# Autodesk Inventor assembly: 5267300 AEN-S-6-5-I-A---(0_high)
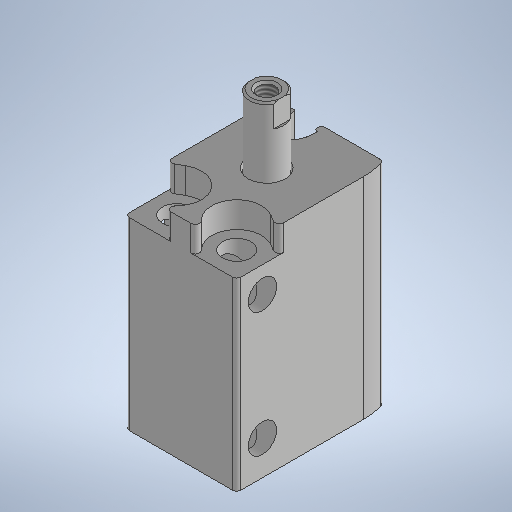
[picture p0: Inventor's stored thumbnail of the model, 512x512]
Saved by Autodesk Inventor 2025.2 (Build 292293000, 293)
## iProperties
Category: PARTsolutions
Company: FESTO
Created: 2025-06-16
Part Number: 5267300 AEN-S-6-5-I-A---(0_high)
Catalog Web Link: www.cadenas.de
Description: AEN-S-Compact cylinder
Vendor: FESTO
Document SubType Name: Assembly
Designer: psAdmin
Manufacturer: FESTO
Mass: 10.9 g
Surface Area: 34.4822 cm^2
Volume: 4.48385 cm^3
Density: 2.43095 g/cm^3
PSOL_IDENT_0: {ATYP=ASSISTANT},{DATA=script=$CADENAS_DATA/23d-libs/festo/webfesto.vbb&M_FAMILY=AEN&M_GROUP=01&M_PA
PSOL_IDENT_1: RTNO=5267300&IDCODE1=AEN-S-6-5-I-A&IDCODE2=&customer_number_cns=&MATES=1&LOD=HI&LOCKERP=0&SINGLEPART=
PSOL_IDENT_2: 1}
NB: 5267300 AEN-S-6-5-I-A---(0_high)
NN: AEN-S
NT: Compact cylinder
NBSYN: $TNR. $TYP.---($HUBST._$LODLEVEL.)
LINA: 5267300 AEN-S-6-5-I-A
CATALOG: Festo
TNR: 5267300
TYP: AEN-S-6-5-I-A
LODLEVEL: High
KDM: 6
HUB: 5
HUBST: 0
GA: I
DAF: P
AFF: A
A: 0
AF: 5
BG: 0
D1: 5.8
D2: 3.3
DA: 0
E1: 13
E2: 17.5
EE: M3
KF: M2.5
KK: -
L3: 10
L4: 7
LA: 0
MM: 4
P1: 6
P2: 4
P3: 3
PL1: 7
PL2: 3
RR: 0
RT: -
SF: 3.5
T: 3
T4: 0
TG: 7
WH: 3
WL: 2.7
ZA: 24.5
ZB: 27.5
CNSMASSEXACT: 0.0109
GTIN: 4052568422400
SUPPLIER: FESTO
ARTICLENO: 5267300 AEN-S-6-5-I-A---(0_high)
BOMINFO: 5267300 AEN-S-6-5-I-A
CREATOR: CADENAS GmbH
Title: 5267300 AEN-S-6-5-I-A
Author: Cadenas PARTsolutions
Comments: Compact cylinder
## Documents named in this file (3)
- C:\Users\Jakob\Documents\Kooperatives Studium HHN\Studium\3. Semester\CAD_Konstruktion - Schillo Paspa\Festo\AIS2024\5267300 AEN-S-6-5-I-A---(0_high).iam
- C:\Users\Jakob\Documents\Kooperatives Studium HHN\Studium\3. Semester\CAD_Konstruktion - Schillo Paspa\Festo\AIS2024\5267300 AEN-S-6-5-I-A---(highH).ipt
- C:\Users\Jakob\Documents\Kooperatives Studium HHN\Studium\3. Semester\CAD_Konstruktion - Schillo Paspa\Festo\AIS2024\5267300 AEN-S-6-5-I-A---(highP).ipt
## Components (2 placed, 2 different names)
1. 5267300 AEN-S-6-5-I-A---(highH):1 — TO_P_XY@1 <-> ANBAU_XY@2, TO_P_Z@1 <-> ANBAU_Z@2, TO_P_YZ@1 <-> ANBAU_YZ@2
2. 5267300 AEN-S-6-5-I-A---(highP):1 — TO_P_XY@1 <-> ANBAU_XY@2, TO_P_Z@1 <-> ANBAU_Z@2, TO_P_YZ@1 <-> ANBAU_YZ@2
## Relationships (3: Mate 2, Angle 1)
- TO_P_XY@1 <-> ANBAU_XY@2 [Mate]: 5267300 AEN-S-6-5-I-A---(highH):1 ↔ 5267300 AEN-S-6-5-I-A---(highP):1
- TO_P_Z@1 <-> ANBAU_Z@2 [Mate]: 5267300 AEN-S-6-5-I-A---(highH):1 ↔ 5267300 AEN-S-6-5-I-A---(highP):1
- TO_P_YZ@1 <-> ANBAU_YZ@2 [Angle] (0 deg): 5267300 AEN-S-6-5-I-A---(highH):1 ↔ 5267300 AEN-S-6-5-I-A---(highP):1
